# Autodesk Inventor assembly: Bottle 5mm thk parts
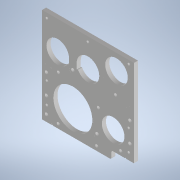
[picture p0: Inventor's stored thumbnail of the model, 180x180]
Saved by Autodesk Inventor 2021 (Build 250183000, 183)
## iProperties
Created: 2020-08-19
Part Number: Bottle 5mm thk parts
Document SubType Name: Assembly
Designer: jgray
Author: jgray
## Documents named in this file (4)
- M:\Printed Electronics\Gas Sensors\Prototypes\Prototype II -Cartridge Reader V3\Bottle 5mm thk parts.iam
- M:\Printed Electronics\Gas Sensors\Prototypes\Prototype II -Cartridge Reader V3\Bottle layout.ipt
- M:\Printed Electronics\Gas Sensors\Prototypes\Prototype II -Cartridge Reader V3\Bottle layout pt3.ipt
- M:\Printed Electronics\Gas Sensors\Prototypes\Prototype II -Cartridge Reader V3\Bottle layout pt2.ipt
## Components (3 placed, 3 different names)
1. Bottle layout:1 — Flush:2, Flush:3, Flush:4, Flush:5
2. Bottle layout pt3:1 — Flush:5
3. Bottle layout pt2:1 — Flush:4
## Relationships (11: Mate 6, Flush 5)
- [Flush]: Bottle layout:1 ↔ Bottle layout pt2:1
- [Mate]: Bottle layout:1 ↔ Bottle layout pt2:1
- [Mate]: Bottle layout pt3:1 ↔ Bottle layout pt2:1
- [Mate]: Bottle layout:1 ↔ Bottle layout pt2:1
- [Mate]: Bottle layout:1 ↔ Bottle layout pt2:1
- [Mate]: Bottle layout pt3:1 ↔ Bottle layout pt2:1
- [Mate]: Bottle layout pt3:1 ↔ Bottle layout pt2:1
- Flush:2: Bottle layout:1
- Flush:3: Bottle layout:1
- Flush:4: Bottle layout:1 ↔ Bottle layout pt2:1
- Flush:5: Bottle layout:1 ↔ Bottle layout pt3:1
## Named parameters: d0_d1 = 0 mm, d1_d2 = 0 mm, d2_d3 = 0 mm
